# Autodesk Inventor assembly: diseñoAdhesionDron
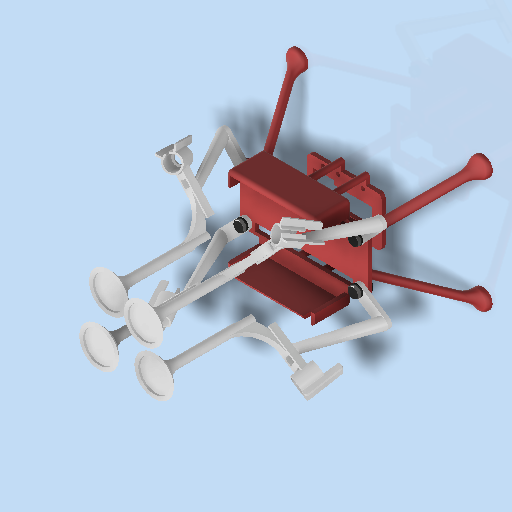
[picture p0: Inventor's stored thumbnail of the model, 512x512]
Saved by Autodesk Inventor 2025.3 (Build 293356030, 356C)
## iProperties
Created: 2025-09-10
Part Number: diseñoAdhesionDron
Document SubType Name: Assembly
Designer: Lenovo
Author: Lenovo
## iProperties of the stored document 7mm motor mount PART2 (draft2).ipt
Created: 2015-06-29
Part Number: 7mm motor mount PART2 (draft2)
Material: Nylon 101
Document SubType Name: Modeling
Designer: Lenovo
Density: 1.15 g/cm^3
Appearance: Valor por defecto
Author: Lenovo
## iProperties of the stored document SupportRASPIwithBattery(Act4).ipt
Created: 2025-08-31
Part Number: SupportRASPIwithBattery(Act4)
Material: Genérico
Document SubType Name: Modeling
Designer: Lenovo
Density: 1 g/cm^3
Appearance: Valor por defecto
Sending System: Autodesk Inventor 2026
Preprocessor: ST-DEVELOPER v20.1
Title: SupportRASPIwithBattery(Act4).stp
Author: s7eep
## iProperties of the stored document Rotor(Esfuerzos).iam
Created: 2025-09-01
Part Number: Rotor(Esfuerzos)
Document SubType Name: Assembly
Designer: Lenovo
Sending System: Autodesk Inventor 2026
Preprocessor: ST-DEVELOPER v20.1
Title: Rotor(Esfuerzos).stp
Author: s7eep
## iProperties of the stored document 7mm motor mount PART2 (draft2).ipt
Created: 2015-06-29
Part Number: 7mm motor mount PART2 (draft2)
Material: Nylon 101
Document SubType Name: Modeling
Designer: Lenovo
Density: 1.15 g/cm^3
Appearance: Valor por defecto
Author: Lenovo
## iProperties of the stored document 7mm motor mount PART1 (edited).ipt
Created: 2015-06-29
Part Number: 7mm motor mount PART1 (edited)
Material: Nylon 101
Document SubType Name: Modeling
Designer: Lenovo
Density: 1.15 g/cm^3
Appearance: Valor por defecto
Author: Lenovo
## iProperties of the stored document Rotor2(Esfuerzos).iam
Created: 2025-09-10
Part Number: Rotor2(Esfuerzos)
Document SubType Name: Assembly
Designer: Lenovo
Sending System: Autodesk Inventor 2026
Preprocessor: ST-DEVELOPER v20.1
Title: Rotor2(Esfuerzos).stp
Author: s7eep
## iProperties of the stored document 7mm motor mount PART1 (edited).ipt
Created: 2015-06-29
Part Number: 7mm motor mount PART1 (edited)
Material: Nylon 101
Document SubType Name: Modeling
Designer: Lenovo
Density: 1.15 g/cm^3
Appearance: Valor por defecto
Author: Lenovo
## Documents named in this file (14)
- D:\marit\Documents\PLANOS DANY\Nueva carpeta (3)\diseñoAdhesionDron.iam
- **D:\marit\Documents\PLANOS DANY\Nueva carpeta (3)\diseñoAdhesionDron.iam*LocalDocs*xAaaaaucaAaaaaaaaAaaaaaal0a*SupportRASPIwithBattery(Act4).ipt
- **D:\marit\Documents\PLANOS DANY\Nueva carpeta (3)\diseñoAdhesionDron.iam*LocalDocs*xAaaaqjdaAaaaaaaaAaaaqqs5Ug*Rotor(Esfuerzos).iam
- D:\marit\Documents\PLANOS DANY\Nueva carpeta (3)\ISO 7091 - ST 2.5 - 100 HV.ipt
- D:\marit\Documents\PLANOS DANY\Nueva carpeta (3)\ISO 4017 - M2.5 x 6 - ISO.ipt
- D:\marit\Documents\PLANOS DANY\Nueva carpeta (3)\ISO 4036 - M2.5(2).ipt
- **D:\marit\Documents\PLANOS DANY\Nueva carpeta (3)\diseñoAdhesionDron.iam*LocalDocs*xAaaaqodaAaaaaaaaAaaaaqg1Ta*Rotor2(Esfuerzos).iam
- D:\marit\Documents\PLANOS DANY\Nueva carpeta (3)\SupportRASPIwithBattery(Act4).stp
- D:\marit\Documents\PLANOS DANY\Nueva carpeta (3)\Rotor(Esfuerzos).stp
- D:\marit\Documents\PLANOS DANY\Nueva carpeta (3)\Rotor2(Esfuerzos).stp
- **D:\marit\Documents\PLANOS DANY\Nueva carpeta (3)\diseñoAdhesionDron.iam*LocalDocs*xAaaaq4daAaaaaaaaAaaaa4vk2h*7mm motor mount PART2 (draft2).ipt
- **D:\marit\Documents\PLANOS DANY\Nueva carpeta (3)\diseñoAdhesionDron.iam*LocalDocs*xAaaaqsaaAaaaaaaaAaaaq4sqCf*7mm motor mount PART1 (edited).ipt
- **D:\marit\Documents\PLANOS DANY\Nueva carpeta (3)\diseñoAdhesionDron.iam*LocalDocs*xAaaaq4daAaaaaaaaAaaaa4vkLh*7mm motor mount PART2 (draft2).ipt
- **D:\marit\Documents\PLANOS DANY\Nueva carpeta (3)\diseñoAdhesionDron.iam*LocalDocs*xAaaaqsaaAaaaaaaaAaaaq4sqTf*7mm motor mount PART1 (edited).ipt
## Components (17 placed, 6 different names)
1. SupportRASPIwithBattery(Act4):1 — Insertar:2, Insertar:3, Coincidencia:4, Insertar:7, Insertar:12, Insertar:14, Insertar:15, Insertar:16
2. Rotor(Esfuerzos):2 [sub-assembly] — Insertar:2, Insertar:8
3. Rotor(Esfuerzos):4 [sub-assembly] — Insertar:3, Insertar:13
4. ISO 7091 ST 2.5 - 100 HV:1 — Insertar:5
5. ISO 4017 M2.5 x 6:1 — Insertar:5
6. ISO 4036 M2.5:1 — Coincidencia:4
7. ISO 7091 ST 2.5 - 100 HV:2 — Insertar:8
8. ISO 4017 M2.5 x 6:2
9. ISO 4036 M2.5:2 — Insertar:7
10. ISO 7091 ST 2.5 - 100 HV:3
11. ISO 4017 M2.5 x 6:3
12. ISO 4036 M2.5:3 — Insertar:12
13. ISO 7091 ST 2.5 - 100 HV:4 — Insertar:13
14. ISO 4017 M2.5 x 6:4
15. ISO 4036 M2.5:4 — Insertar:14
16. Rotor2(Esfuerzos):1 [sub-assembly] — Insertar:15
17. Rotor2(Esfuerzos):2 [sub-assembly] — Insertar:16
## Relationships (14: Insert 13, Mate 1)
- Insertar:2: SupportRASPIwithBattery(Act4):1 ↔ Rotor(Esfuerzos):2
- Insertar:3: SupportRASPIwithBattery(Act4):1 ↔ Rotor(Esfuerzos):4
- Insertar:5: ISO 7091 ST 2.5 - 100 HV:1 ↔ ISO 4017 M2.5 x 6:1
- Coincidencia:4 [Mate]: SupportRASPIwithBattery(Act4):1 ↔ ISO 4036 M2.5:1
- [Insert]: ISO 7091 ST 2.5 - 100 HV:2 ↔ ISO 4017 M2.5 x 6:2
- Insertar:7: SupportRASPIwithBattery(Act4):1 ↔ ISO 4036 M2.5:2
- Insertar:8: Rotor(Esfuerzos):2 ↔ ISO 7091 ST 2.5 - 100 HV:2
- [Insert]: ISO 7091 ST 2.5 - 100 HV:3 ↔ ISO 4017 M2.5 x 6:3
- [Insert]: ISO 7091 ST 2.5 - 100 HV:4 ↔ ISO 4017 M2.5 x 6:4
- Insertar:12: SupportRASPIwithBattery(Act4):1 ↔ ISO 4036 M2.5:3
- Insertar:13: Rotor(Esfuerzos):4 ↔ ISO 7091 ST 2.5 - 100 HV:4
- Insertar:14: SupportRASPIwithBattery(Act4):1 ↔ ISO 4036 M2.5:4
- Insertar:15: SupportRASPIwithBattery(Act4):1 ↔ Rotor2(Esfuerzos):1
- Insertar:16: SupportRASPIwithBattery(Act4):1 ↔ Rotor2(Esfuerzos):2
## Named parameters: d11_d6 = 0 mm, d12_d7 = 0 mm, d13_d8 = 0 mm, d16_d11_d6 = 0 mm, d17_d12_d7 = 0 mm, d18_d13_d8 = 0 mm, d19_d11_d6 = 0 mm, d20_d12_d7 = 0 mm, d21_d13_d8 = 0 mm
